# Autodesk Inventor assembly: BRTIRUS2110A 六轴机器人模型（11版本）
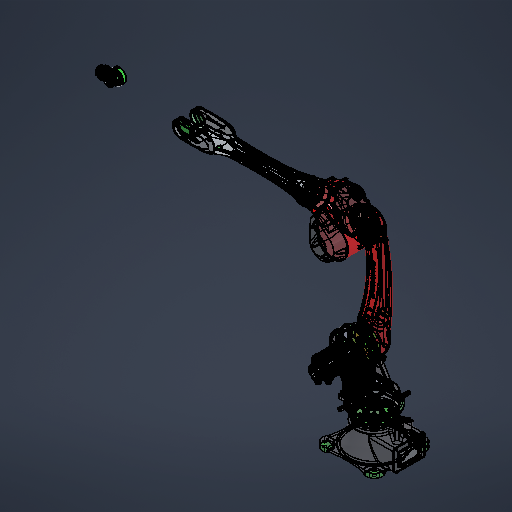
[picture p0: Inventor's stored thumbnail of the model, 512x512]
Saved by Autodesk Inventor 2025.1 (Build 291241000, 241)
## iProperties
Created: 2023-03-18
Part Number: BRTIRUS2110A 六轴机器人模型（11版本）
Description: STEP AP214
Document SubType Name: Assembly
Designer: Якимов С.Е.
Sending System: SolidWorks 2014
Preprocessor: SwSTEP 2.0
Title: BRTIRUS2110A ÁùÖá»úÆ÷ÈËÄ£ÐÍ£¨11°æ±¾£©.STEP
Revision Number: ÈÎºÎ
## Documents named in this file (8)
- C:\Users\YakimovSE\Desktop\BRTIRUS2110A\1. 机器人模型\BRTIRUS2110A 六轴机器人模型（11版本）\BRTIRUS2110A 六轴机器人模型（11版本）\BRTIRUS2110A 六轴机器人模型（11版本）.iam
- C:\Users\YakimovSE\Desktop\BRTIRUS2110A\1. 机器人模型\BRTIRUS2110A 六轴机器人模型（11版本）\BRTIRUS2110A 六轴机器人模型（11版本）\PAR6US21A001 µ××ù.ipt
- C:\Users\YakimovSE\Desktop\BRTIRUS2110A\1. 机器人模型\BRTIRUS2110A 六轴机器人模型（11版本）\BRTIRUS2110A 六轴机器人模型（11版本）\PAR6US21B001 µÚ2Öá×°Åä²¿.ipt
- C:\Users\YakimovSE\Desktop\BRTIRUS2110A\1. 机器人模型\BRTIRUS2110A 六轴机器人模型（11版本）\BRTIRUS2110A 六轴机器人模型（11版本）\PAR6US18C001 µÚ3Öá´ó±Û×°Åä²¿.ipt
- C:\Users\YakimovSE\Desktop\BRTIRUS2110A\1. 机器人模型\BRTIRUS2110A 六轴机器人模型（11版本）\BRTIRUS2110A 六轴机器人模型（11版本）\PAR6US21D001 µÚ4Öá×°Åä²¿.ipt
- C:\Users\YakimovSE\Desktop\BRTIRUS2110A\1. 机器人模型\BRTIRUS2110A 六轴机器人模型（11版本）\BRTIRUS2110A 六轴机器人模型（11版本）\PAR6US21E001 µÚ5Öá×°Åä²¿.ipt
- C:\Users\YakimovSE\Desktop\BRTIRUS2110A\1. 机器人模型\BRTIRUS2110A 六轴机器人模型（11版本）\BRTIRUS2110A 六轴机器人模型（11版本）\PAR6US21F001 ÁùÖá×°ÅäÌå.ipt
- C:\Users\YakimovSE\Desktop\BRTIRUS2110A\1. 机器人模型\BRTIRUS2110A 六轴机器人模型（11版本）\BRTIRUS2110A 六轴机器人模型（11版本）\PAR6US21F002 Ä©¶Ë.ipt
## Components (7 placed, 7 different names)
1. PAR6US21A001 µ××ù_1 — Жесткий:1
2. PAR6US21B001 µÚ2Öá×°Åä²¿_2 — Жесткий:1, Жесткий:2
3. PAR6US18C001 µÚ3Öá´ó±Û×°Åä²¿_3 — Жесткий:2, Жесткий:3
4. PAR6US21D001 µÚ4Öá×°Åä²¿_4 — Жесткий:3, Жесткий:4
5. PAR6US21E001 µÚ5Öá×°Åä²¿_5 — Жесткий:4
6. PAR6US21F001 ÁùÖá×°ÅäÌå_6
7. PAR6US21F002 Ä©¶Ë_7
## Relationships (4: WeldJoint 4)
- Жесткий:1 [WeldJoint]: PAR6US21A001 µ××ù_1 ↔ PAR6US21B001 µÚ2Öá×°Åä²¿_2
- Жесткий:2 [WeldJoint]: PAR6US21B001 µÚ2Öá×°Åä²¿_2 ↔ PAR6US18C001 µÚ3Öá´ó±Û×°Åä²¿_3
- Жесткий:3 [WeldJoint]: PAR6US18C001 µÚ3Öá´ó±Û×°Åä²¿_3 ↔ PAR6US21D001 µÚ4Öá×°Åä²¿_4
- Жесткий:4 [WeldJoint]: PAR6US21D001 µÚ4Öá×°Åä²¿_4 ↔ PAR6US21E001 µÚ5Öá×°Åä²¿_5
